# Autodesk Inventor assembly: Robot - Blue Alliance
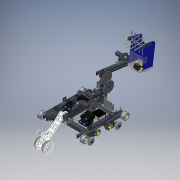
[picture p0: Inventor's stored thumbnail of the model, 180x180]
Saved by Autodesk Inventor 2016 (Build 200138000, 138)
## iProperties
Created: 2015-12-13
Part Number: Robot - Blue Alliance
Document SubType Name: Assembly
Designer: tbloo
Author: tbloo
## Documents named in this file (39)
- C:\Users\TimB\Documents\GitHub\phi_robotics\3d-models\FTC_Tetrix_KOP_Block_Party\Tim Bloot Designs\JAr JaR Bot\Robot - Blue Alliance.iam
- C:\Users\TimB\Documents\GitHub\phi_robotics\3d-models\FTC_Tetrix_KOP_Block_Party\Tim Bloot Designs\Base Plate.ipt
- C:\Users\TimB\Documents\GitHub\phi_robotics\3d-models\FTC_Tetrix_KOP_Block_Party\Tetrix_Kit_FTC\Autodesk Inventor Files\tetrix_c_channel-3.ipt
- C:\Users\TimB\Documents\GitHub\phi_robotics\3d-models\FTC_Tetrix_KOP_Block_Party\Tetrix_Kit_FTC\Autodesk Inventor Files\tetrix_c_channel-2.ipt
- C:\Users\TimB\Documents\GitHub\phi_robotics\3d-models\FTC_Tetrix_KOP_Block_Party\Tetrix_Kit_FTC\Autodesk Inventor Files\tetrix_motor_mount-old.ipt
- C:\Users\TimB\Documents\GitHub\phi_robotics\3d-models\FTC_Tetrix_KOP_Block_Party\Tetrix_Kit_FTC\Autodesk Inventor Files\tetrix_motor.iam
- C:\Users\TimB\Documents\GitHub\phi_robotics\3d-models\FTC_Tetrix_KOP_Block_Party\Tetrix_Kit_FTC\Autodesk Inventor Files\tetrix_bushing.ipt
- C:\Users\TimB\Documents\GitHub\phi_robotics\3d-models\FTC_Tetrix_KOP_Block_Party\Tim Bloot Designs\JAr JaR Bot\Tread Wheel Assembly.iam
- C:\Users\TimB\Documents\GitHub\phi_robotics\3d-models\FTC_Tetrix_KOP_Block_Party\Tetrix_Kit_FTC\Autodesk Inventor Files\tetrix_motor_controller.ipt
- C:\Users\TimB\Documents\GitHub\phi_robotics\3d-models\FTC_Tetrix_KOP_Block_Party\Tetrix_Kit_FTC\Autodesk Inventor Files\tetrix_c_channel-round.ipt
- C:\Users\TimB\Documents\GitHub\phi_robotics\3d-models\FTC_Tetrix_KOP_Block_Party\Tetrix_Kit_FTC\Autodesk Inventor Files\tetrix_c_channel-1.ipt
- C:\Users\TimB\Documents\GitHub\phi_robotics\3d-models\FTC_Tetrix_KOP_Block_Party\Tim Bloot Designs\JAr JaR Bot\Tread Sproket Gear Assembly 2.iam
- C:\Users\TimB\Documents\GitHub\phi_robotics\3d-models\FTC_Tetrix_KOP_Block_Party\Tim Bloot Designs\JAr JaR Bot\Motor Med Chain gear.iam
- C:\Users\TimB\Documents\GitHub\phi_robotics\3d-models\FTC_Tetrix_KOP_Block_Party\Tim Bloot Designs\JAr JaR Bot\tetrix_angle-144 MM.ipt
- C:\Users\TimB\Documents\GitHub\phi_robotics\3d-models\FTC_Tetrix_KOP_Block_Party\Tim Bloot Designs\JAr JaR Bot\inside Angle beam.ipt
- C:\Users\TimB\Documents\GitHub\phi_robotics\3d-models\FTC_Tetrix_KOP_Block_Party\Tetrix_Kit_FTC\Autodesk Inventor Files\tetrix_739107_2013.ipt
- C:\Users\TimB\Documents\GitHub\phi_robotics\3d-models\FTC_Tetrix_KOP_Block_Party\Tim Bloot Designs\JAr JaR Bot\cut c channel.ipt
- C:\Users\TimB\Documents\GitHub\phi_robotics\3d-models\FTC_Tetrix_KOP_Block_Party\Tetrix_Kit_FTC\Autodesk Inventor Files\tetrix_c_channel-4.ipt
- C:\Users\TimB\Documents\GitHub\phi_robotics\3d-models\FTC_Tetrix_KOP_Block_Party\Tetrix_Kit_FTC\Autodesk Inventor Files\tetrix_inside_corner_bracket.ipt
- C:\Users\TimB\Documents\GitHub\phi_robotics\3d-models\FTC_Tetrix_KOP_Block_Party\Tetrix_Kit_FTC\Autodesk Inventor Files\tetrix_worm_gear-p3.ipt
- C:\Users\TimB\Documents\GitHub\phi_robotics\3d-models\FTC_Tetrix_KOP_Block_Party\Tetrix_Kit_FTC\Autodesk Inventor Files\tetrix_servo_controller.ipt
- C:\Users\TimB\Documents\GitHub\phi_robotics\3d-models\FTC_Tetrix_KOP_Block_Party\Tim Bloot Designs\JAr JaR Bot\Blue Alliance Arm.iam
- C:\Users\TimB\Documents\GitHub\phi_robotics\3d-models\FTC_Tetrix_KOP_Block_Party\Tetrix_Kit_FTC\Autodesk Inventor Files\tetrix_standoff_post-1in.ipt
- C:\Users\TimB\Documents\GitHub\phi_robotics\3d-models\FTC_Tetrix_KOP_Block_Party\Tetrix_Kit_FTC\Autodesk Inventor Files\tetrix_axle_lock.iam
- C:\Users\TimB\Documents\GitHub\phi_robotics\3d-models\FTC_Tetrix_KOP_Block_Party\Tetrix_Kit_FTC\Autodesk Inventor Files\tetrix_gear-large.ipt
- C:\Users\TimB\Documents\GitHub\phi_robotics\3d-models\FTC_Tetrix_KOP_Block_Party\Tetrix_Kit_FTC\Autodesk Inventor Files\tetrix_gear-small.ipt
- C:\Users\TimB\Documents\GitHub\phi_robotics\3d-models\FTC_Tetrix_KOP_Block_Party\Tetrix_Kit_FTC\Autodesk Inventor Files\tetrix_axle_spacer_mount.ipt
- C:\Users\TimB\Documents\GitHub\phi_robotics\3d-models\FTC_Tetrix_KOP_Block_Party\Tetrix_Kit_FTC\Autodesk Inventor Files\tetrix_axle.ipt
- C:\Users\TimB\Documents\GitHub\phi_robotics\3d-models\FTC_Tetrix_KOP_Block_Party\Tetrix_Kit_FTC\Autodesk Inventor Files\tetrix_739092_2012.iam
- C:\Users\TimB\Documents\GitHub\phi_robotics\3d-models\FTC_Tetrix_KOP_Block_Party\Tetrix_Kit_FTC\Autodesk Inventor Files\tetrix_gear-med.ipt
- C:\Users\TimB\Documents\GitHub\phi_robotics\3d-models\FTC_Tetrix_KOP_Block_Party\Tim Bloot Designs\JAr JaR Bot\WheelieBar Blue Alliance.iam
- C:\Users\TimB\Documents\GitHub\phi_robotics\3d-models\FTC_Tetrix_KOP_Block_Party\Tetrix_Kit_FTC\Autodesk Inventor Files\tetrix_chain_gear-16t.ipt
- C:\Users\TimB\Documents\GitHub\phi_robotics\3d-models\FTC_Tetrix_KOP_Block_Party\Tetrix_Kit_FTC\Autodesk Inventor Files\tetrix_maxle_lock.iam
- C:\Users\TimB\Documents\GitHub\phi_robotics\3d-models\FTC_Tetrix_KOP_Block_Party\Tim Bloot Designs\Legacy Module.ipt
- C:\Users\TimB\Documents\GitHub\phi_robotics\3d-models\FTC_Tetrix_KOP_Block_Party\Tetrix_Kit_FTC\Autodesk Inventor Files\tetrix_batterypack.ipt
- C:\Users\TimB\Documents\GitHub\phi_robotics\3d-models\FTC_Tetrix_KOP_Block_Party\Tim Bloot Designs\Flag Mount.ipt
- C:\Users\TimB\Documents\GitHub\phi_robotics\3d-models\FTC_Tetrix_KOP_Block_Party\Tim Bloot Designs\Phone Mount 2.ipt
- C:\Users\TimB\Documents\GitHub\phi_robotics\3d-models\FTC_Tetrix_KOP_Block_Party\Tetrix_Kit_FTC\Autodesk Inventor Files\tetrix_739280_2013.ipt
- C:\Users\TimB\Documents\GitHub\phi_robotics\3d-models\FTC_Tetrix_KOP_Block_Party\Tetrix_Kit_FTC\Autodesk Inventor Files\tetrix_servo_body.ipt
## Components (128 placed, 38 different names)
1. Base Plate:1 — Rigid:117, Rigid:121, Rigid:127, Rigid:137, Rigid:140, Rigid:157, Rigid:162, Rigid:161, Rigid:163, Rigid:164, Mate:1
2. tetrix_c_channel-3:4 — Rigid:110, Rigid:122, Rigid:126, Rigid:142, Rigid:160
3. tetrix_c_channel-2:13 — Rigid:64, Rigid:111, Rigid:141
4. tetrix_c_channel-2:15 — Rigid:109, Rigid:143, Rigid:191
5. tetrix_c_channel-2:16 — Rigid:124, Rigid:148
6. tetrix_motor_mount-old:6
7. tetrix_motor:5 [sub-assembly] — Rigid:91
8. Tread Wheel Assembly:5 [sub-assembly]
9. Tread Wheel Assembly:6 [sub-assembly]
10. tetrix_c_channel-round:1 — Rigid:64, Rigid:65
11. tetrix_c_channel-1:1 — Rigid:65, Rotational:33, Rotational:34
12. tetrix_bushing:13 — Rotational:33, Rotational:42
13. tetrix_bushing:14 — Rotational:34
14. tetrix_c_channel-2:18 — Rigid:123, Rigid:125
15. tetrix_motor_mount-old:8 — Rotational:41
16. tetrix_c_channel-round:3
17. tetrix_c_channel-1:3
18. tetrix_bushing:17
19. tetrix_bushing:18 — Rotational:43
20. tetrix_motor:6 [sub-assembly] — Rotational:41, Rigid:92
21. Tread Sproket Gear Assembly 2:1 [sub-assembly] — Rotational:42
22. Tread Sproket Gear Assembly 2:2 [sub-assembly] — Rotational:43
23. Motor Med Chain gear:1 [sub-assembly] — Rigid:92
24. Motor Med Chain gear:2 [sub-assembly] — Rigid:91
25. tetrix_c_channel-3:5 — Rigid:116, Rigid:133, Rigid:136, Rigid:139
26. tetrix_c_channel-2:19 — Rigid:115, Rigid:135
27. tetrix_c_channel-2:20 — Rigid:134, Rigid:147
28. tetrix_c_channel-2:21 — Rigid:131, Rigid:144, Rigid:192
29. tetrix_motor_mount-old:9
30. tetrix_motor:7 [sub-assembly]
31. Tread Wheel Assembly:7 [sub-assembly]
32. Tread Wheel Assembly:8 [sub-assembly]
33. tetrix_c_channel-round:4
34. tetrix_c_channel-1:4
35. tetrix_bushing:19
36. tetrix_bushing:20
37. tetrix_c_channel-2:22 — Rigid:132, Rigid:138
38. tetrix_motor_mount-old:10
39. tetrix_c_channel-round:5
40. tetrix_c_channel-1:5
41. tetrix_bushing:21
42. tetrix_bushing:22
43. tetrix_motor:8 [sub-assembly]
44. Tread Sproket Gear Assembly 2:3 [sub-assembly]
45. Tread Sproket Gear Assembly 2:4 [sub-assembly]
46. Motor Med Chain gear:3 [sub-assembly]
47. Motor Med Chain gear:4 [sub-assembly]
48. tetrix_angle-144 MM:1 — Rigid:109, Rigid:110, Rigid:111
49. inside Angle beam:1 — Rigid:137, Rigid:138, Rigid:139
50. inside Angle beam:2 — Rigid:115, Rigid:116, Rigid:117
51. inside Angle beam:3 — Rigid:140, Rigid:141, Rigid:142, Mate:2
52. inside Angle beam:4 — Rigid:121, Rigid:122, Rigid:123
53. tetrix_angle-144 MM:2 — Rigid:124, Rigid:125, Rigid:126
54. tetrix_739107_2013:1 — Rigid:129
55. tetrix_739107_2013:2 — Rigid:128, Rigid:130
56. tetrix_motor_controller:1 — Rigid:127, Rigid:128, Rigid:129
57. tetrix_motor_controller:2 — Rigid:130
58. tetrix_angle-144 MM:3 — Rigid:134, Rigid:135, Rigid:136
59. tetrix_angle-144 MM:4 — Rigid:131, Rigid:132, Rigid:133
60. cut c channel:1 — Rigid:149, Rigid:151, Rigid:152, Rigid:172, Rotational:61, Rotational:62, Rotational:66, Rotational:67, Rigid:182, Rotational:75
61. cut c channel:2 — Rigid:143, Rigid:144, Rigid:151, Rigid:153, Mate:3, Rigid:188
62. tetrix_c_channel-4:1 — Rigid:145, Rigid:146, Rigid:150
63. tetrix_inside_corner_bracket:1 — Rigid:145, Rigid:148
64. tetrix_inside_corner_bracket:2 — Rigid:146, Rigid:147
65. tetrix_worm_gear-p3:1 — Rigid:149, Rigid:150
66. tetrix_c_channel-4:2 — Rigid:152, Rigid:153, Rotational:54, Rotational:55, Rotational:58, Rotational:59, Rigid:171, Rigid:189
67. tetrix_739107_2013:3 — Rigid:158
68. tetrix_739107_2013:4 — Rigid:159
69. tetrix_motor_controller:3 — Rigid:157
70. tetrix_servo_controller:1 — Rigid:158, Rigid:159
71. Blue Alliance Arm:1 [sub-assembly] — Rigid:186
72. tetrix_c_channel-1:6 — Rigid:160
73. tetrix_standoff_post-1in:1 — Rigid:162
74. tetrix_standoff_post-1in:2 — Rigid:163, Rigid:187
75. tetrix_standoff_post-1in:3 — Rigid:164
76. tetrix_standoff_post-1in:4 — Rigid:161
77. tetrix_bushing:23 — Rotational:54
78. tetrix_bushing:24 — Rotational:55, Rotational:56
79. tetrix_axle_lock:1 [sub-assembly] — Rigid:165, Rotational:56
80. tetrix_gear-large:1 — Rigid:165, Rigid:186
81. tetrix_gear-large:2 — Rigid:166
82. tetrix_gear-small:1 — Rigid:167, Rigid:168
83. tetrix_axle_spacer_mount:1 — Rigid:166, Rigid:167, Rotational:57
84. tetrix_axle_lock:2 [sub-assembly] — Rigid:168, Rigid:170
85. tetrix_bushing:25 — Rotational:57
86. tetrix_bushing:26 — Rotational:58
87. tetrix_bushing:27 — Rotational:59, Rotational:60
88. tetrix_axle:1 — Rigid:169, Rigid:170
89. tetrix_739092_2012:1 [sub-assembly] — Rigid:169, Rotational:60
90. tetrix_motor_mount-old:11 — Rigid:171, Rotational:64
91. tetrix_motor_mount-old:12 — Rigid:173, Rotational:65
92. tetrix_c_channel-round:6 — Rigid:172, Rigid:173
93. tetrix_gear-large:3 — Rigid:177
94. tetrix_axle_spacer_mount:2 — Rigid:175, Rigid:176
95. tetrix_gear-med:1 — Rigid:175
96. tetrix_bushing:28 — Rigid:176, Rigid:179
97. tetrix_739092_2012:2 [sub-assembly] — Rigid:178, Rigid:179
98. tetrix_axle_lock:3 [sub-assembly] — Rigid:177, Rotational:63
99. tetrix_axle:2 — Rigid:178, Rigid:180
100. tetrix_bushing:29 — Rotational:62
101. tetrix_bushing:30 — Rotational:61, Rotational:63
102. tetrix_739092_2012:3 [sub-assembly] — Rigid:180
103. tetrix_motor:9 [sub-assembly] — Rotational:64
104. tetrix_motor:10 [sub-assembly] — Rotational:65
105. tetrix_bushing:31 — Rotational:67, Rotational:70
106. tetrix_bushing:32 — Rotational:66
107. tetrix_c_channel-round:7 — Rigid:182, Rigid:183
108. tetrix_motor_mount-old:13 — Rigid:183, Rotational:69
109. tetrix_motor:11 [sub-assembly] — Rotational:69, Rigid:185
110. tetrix_maxle_lock:1 [sub-assembly] — Rigid:185, Rigid:194
111. WheelieBar Blue Alliance:1 [sub-assembly] — Rotational:70
112. Legacy Module:1 — Rigid:187
113. tetrix_batterypack:1 — Mate:1, Mate:2, Mate:3
114. Flag Mount:1 — Rigid:190
115. Phone Mount 2:1 — Rigid:188
116. tetrix_c_channel-1:7 — Rigid:189, Rigid:190
117. tetrix_739280_2013:1 — Rigid:191, Rotational:72, Rigid:193
118. tetrix_739280_2013:2 — Rigid:192, Rotational:71
119. tetrix_bushing:33 — Rotational:71
120. tetrix_bushing:34 — Rotational:72
121. tetrix_servo_body:1 — Rigid:193
122. tetrix_gear-small:2 — Rigid:194
123. tetrix_gear-med:3
124. tetrix_chain_gear-16t:2
125. tetrix_axle_lock:4 [sub-assembly]
126. tetrix_axle:3
127. tetrix_bushing:35
128. tetrix_bushing:36 — Rotational:75
## Relationships (140: WeldJoint 96, RevoluteJoint 41, Mate 3)
- [WeldJoint]: tetrix_c_channel-2:13 ↔ tetrix_motor_mount-old:6
- [RevoluteJoint]: tetrix_motor_mount-old:6 ↔ tetrix_motor:5
- [RevoluteJoint]: tetrix_c_channel-2:15 ↔ Tread Wheel Assembly:5
- [RevoluteJoint]: tetrix_c_channel-2:16 ↔ Tread Wheel Assembly:6
- Rigid:64 [WeldJoint]: tetrix_c_channel-2:13 ↔ tetrix_c_channel-round:1
- Rigid:65 [WeldJoint]: tetrix_c_channel-round:1 ↔ tetrix_c_channel-1:1
- Rotational:33 [RevoluteJoint]: tetrix_c_channel-1:1 ↔ tetrix_bushing:13
- Rotational:34 [RevoluteJoint]: tetrix_c_channel-1:1 ↔ tetrix_bushing:14
- [WeldJoint]: tetrix_c_channel-2:18 ↔ tetrix_motor_mount-old:8
- [WeldJoint]: tetrix_c_channel-2:18 ↔ tetrix_c_channel-round:3
- [WeldJoint]: tetrix_c_channel-round:3 ↔ tetrix_c_channel-1:3
- [RevoluteJoint]: tetrix_c_channel-1:3 ↔ tetrix_bushing:17
- [RevoluteJoint]: tetrix_c_channel-1:3 ↔ tetrix_bushing:18
- Rotational:41 [RevoluteJoint]: tetrix_motor_mount-old:8 ↔ tetrix_motor:6
- Rotational:42 [RevoluteJoint]: tetrix_bushing:13 ↔ Tread Sproket Gear Assembly 2:1
- Rotational:43 [RevoluteJoint]: tetrix_bushing:18 ↔ Tread Sproket Gear Assembly 2:2
- Rigid:91 [WeldJoint]: tetrix_motor:5 ↔ Motor Med Chain gear:2
- Rigid:92 [WeldJoint]: tetrix_motor:6 ↔ Motor Med Chain gear:1
- [WeldJoint]: tetrix_c_channel-2:19 ↔ tetrix_motor_mount-old:9
- [RevoluteJoint]: tetrix_motor_mount-old:9 ↔ tetrix_motor:7
- [RevoluteJoint]: tetrix_c_channel-2:20 ↔ Tread Wheel Assembly:7
- [RevoluteJoint]: tetrix_c_channel-2:21 ↔ Tread Wheel Assembly:8
- [WeldJoint]: tetrix_c_channel-2:19 ↔ tetrix_c_channel-round:4
- [WeldJoint]: tetrix_c_channel-round:4 ↔ tetrix_c_channel-1:4
- [RevoluteJoint]: tetrix_c_channel-1:4 ↔ tetrix_bushing:19
- [RevoluteJoint]: tetrix_c_channel-1:4 ↔ tetrix_bushing:20
- [WeldJoint]: tetrix_c_channel-2:22 ↔ tetrix_motor_mount-old:10
- [WeldJoint]: tetrix_c_channel-2:22 ↔ tetrix_c_channel-round:5
- [WeldJoint]: tetrix_c_channel-round:5 ↔ tetrix_c_channel-1:5
- [RevoluteJoint]: tetrix_c_channel-1:5 ↔ tetrix_bushing:21
- [RevoluteJoint]: tetrix_c_channel-1:5 ↔ tetrix_bushing:22
- [RevoluteJoint]: tetrix_motor_mount-old:10 ↔ tetrix_motor:8
- [RevoluteJoint]: tetrix_bushing:19 ↔ Tread Sproket Gear Assembly 2:3
- [RevoluteJoint]: tetrix_bushing:22 ↔ Tread Sproket Gear Assembly 2:4
- [WeldJoint]: tetrix_motor:7 ↔ Motor Med Chain gear:4
- [WeldJoint]: tetrix_motor:8 ↔ Motor Med Chain gear:3
- Rigid:109 [WeldJoint]: tetrix_c_channel-2:15 ↔ tetrix_angle-144 MM:1
- Rigid:110 [WeldJoint]: tetrix_c_channel-3:4 ↔ tetrix_angle-144 MM:1
- Rigid:111 [WeldJoint]: tetrix_c_channel-2:13 ↔ tetrix_angle-144 MM:1
- Rigid:115 [WeldJoint]: tetrix_c_channel-2:19 ↔ inside Angle beam:2
- Rigid:116 [WeldJoint]: tetrix_c_channel-3:5 ↔ inside Angle beam:2
- Rigid:117 [WeldJoint]: Base Plate:1 ↔ inside Angle beam:2
- Rigid:121 [WeldJoint]: Base Plate:1 ↔ inside Angle beam:4
- Rigid:122 [WeldJoint]: tetrix_c_channel-3:4 ↔ inside Angle beam:4
- Rigid:123 [WeldJoint]: tetrix_c_channel-2:18 ↔ inside Angle beam:4
- Rigid:124 [WeldJoint]: tetrix_c_channel-2:16 ↔ tetrix_angle-144 MM:2
- Rigid:125 [WeldJoint]: tetrix_c_channel-2:18 ↔ tetrix_angle-144 MM:2
- Rigid:126 [WeldJoint]: tetrix_c_channel-3:4 ↔ tetrix_angle-144 MM:2
- Rigid:127 [WeldJoint]: Base Plate:1 ↔ tetrix_motor_controller:1
- Rigid:128 [WeldJoint]: tetrix_739107_2013:2 ↔ tetrix_motor_controller:1
- Rigid:129 [WeldJoint]: tetrix_739107_2013:1 ↔ tetrix_motor_controller:1
- Rigid:130 [WeldJoint]: tetrix_739107_2013:2 ↔ tetrix_motor_controller:2
- Rigid:131 [WeldJoint]: tetrix_c_channel-2:21 ↔ tetrix_angle-144 MM:4
- Rigid:132 [WeldJoint]: tetrix_c_channel-2:22 ↔ tetrix_angle-144 MM:4
- Rigid:133 [WeldJoint]: tetrix_c_channel-3:5 ↔ tetrix_angle-144 MM:4
- Rigid:134 [WeldJoint]: tetrix_c_channel-2:20 ↔ tetrix_angle-144 MM:3
- Rigid:135 [WeldJoint]: tetrix_c_channel-2:19 ↔ tetrix_angle-144 MM:3
- Rigid:136 [WeldJoint]: tetrix_c_channel-3:5 ↔ tetrix_angle-144 MM:3
- Rigid:137 [WeldJoint]: Base Plate:1 ↔ inside Angle beam:1
- Rigid:138 [WeldJoint]: tetrix_c_channel-2:22 ↔ inside Angle beam:1
- Rigid:139 [WeldJoint]: tetrix_c_channel-3:5 ↔ inside Angle beam:1
- Rigid:140 [WeldJoint]: Base Plate:1 ↔ inside Angle beam:3
- Rigid:141 [WeldJoint]: tetrix_c_channel-2:13 ↔ inside Angle beam:3
- Rigid:142 [WeldJoint]: tetrix_c_channel-3:4 ↔ inside Angle beam:3
- Rigid:143 [WeldJoint]: tetrix_c_channel-2:15 ↔ cut c channel:2
- Rigid:144 [WeldJoint]: tetrix_c_channel-2:21 ↔ cut c channel:2
- Rigid:145 [WeldJoint]: tetrix_c_channel-4:1 ↔ tetrix_inside_corner_bracket:1
- Rigid:146 [WeldJoint]: tetrix_c_channel-4:1 ↔ tetrix_inside_corner_bracket:2
- Rigid:147 [WeldJoint]: tetrix_c_channel-2:20 ↔ tetrix_inside_corner_bracket:2
- Rigid:148 [WeldJoint]: tetrix_c_channel-2:16 ↔ tetrix_inside_corner_bracket:1
- Rigid:149 [WeldJoint]: cut c channel:1 ↔ tetrix_worm_gear-p3:1
- Rigid:150 [WeldJoint]: tetrix_c_channel-4:1 ↔ tetrix_worm_gear-p3:1
- Rigid:151 [WeldJoint]: cut c channel:1 ↔ cut c channel:2
- Rigid:152 [WeldJoint]: cut c channel:1 ↔ tetrix_c_channel-4:2
- Rigid:153 [WeldJoint]: cut c channel:2 ↔ tetrix_c_channel-4:2
- [WeldJoint]: tetrix_739107_2013:4 ↔ tetrix_motor_controller:3
- [WeldJoint]: tetrix_739107_2013:3 ↔ tetrix_motor_controller:3
- Rigid:157 [WeldJoint]: Base Plate:1 ↔ tetrix_motor_controller:3
- Rigid:158 [WeldJoint]: tetrix_739107_2013:3 ↔ tetrix_servo_controller:1
- Rigid:159 [WeldJoint]: tetrix_739107_2013:4 ↔ tetrix_servo_controller:1
- Rigid:160 [WeldJoint]: tetrix_c_channel-3:4 ↔ tetrix_c_channel-1:6
- Rigid:162 [WeldJoint]: Base Plate:1 ↔ tetrix_standoff_post-1in:1
- Rigid:161 [WeldJoint]: Base Plate:1 ↔ tetrix_standoff_post-1in:4
- Rigid:163 [WeldJoint]: Base Plate:1 ↔ tetrix_standoff_post-1in:2
- Rigid:164 [WeldJoint]: Base Plate:1 ↔ tetrix_standoff_post-1in:3
- Rotational:54 [RevoluteJoint]: tetrix_c_channel-4:2 ↔ tetrix_bushing:23
- Rotational:55 [RevoluteJoint]: tetrix_c_channel-4:2 ↔ tetrix_bushing:24
- Rigid:165 [WeldJoint]: tetrix_axle_lock:1 ↔ tetrix_gear-large:1
- Rotational:56 [RevoluteJoint]: tetrix_bushing:24 ↔ tetrix_axle_lock:1
- Rigid:166 [WeldJoint]: tetrix_gear-large:2 ↔ tetrix_axle_spacer_mount:1
- Rigid:167 [WeldJoint]: tetrix_gear-small:1 ↔ tetrix_axle_spacer_mount:1
- Rotational:57 [RevoluteJoint]: tetrix_axle_spacer_mount:1 ↔ tetrix_bushing:25
- Rigid:168 [WeldJoint]: tetrix_gear-small:1 ↔ tetrix_axle_lock:2
- Rotational:58 [RevoluteJoint]: tetrix_c_channel-4:2 ↔ tetrix_bushing:26
- Rotational:59 [RevoluteJoint]: tetrix_c_channel-4:2 ↔ tetrix_bushing:27
- Rigid:169 [WeldJoint]: tetrix_axle:1 ↔ tetrix_739092_2012:1
- Rotational:60 [RevoluteJoint]: tetrix_bushing:27 ↔ tetrix_739092_2012:1
- Rigid:170 [WeldJoint] (-41.4 mm): tetrix_axle_lock:2 ↔ tetrix_axle:1
- Rigid:171 [WeldJoint]: tetrix_c_channel-4:2 ↔ tetrix_motor_mount-old:11
- Rigid:172 [WeldJoint]: cut c channel:1 ↔ tetrix_c_channel-round:6
- Rigid:173 [WeldJoint]: tetrix_motor_mount-old:12 ↔ tetrix_c_channel-round:6
- [WeldJoint]: tetrix_gear-large:3 ↔ tetrix_axle_spacer_mount:2
- Rigid:175 [WeldJoint]: tetrix_axle_spacer_mount:2 ↔ tetrix_gear-med:1
- Rigid:176 [WeldJoint]: tetrix_axle_spacer_mount:2 ↔ tetrix_bushing:28
- Rigid:177 [WeldJoint]: tetrix_gear-large:3 ↔ tetrix_axle_lock:3
- Rigid:178 [WeldJoint]: tetrix_739092_2012:2 ↔ tetrix_axle:2
- Rigid:179 [WeldJoint]: tetrix_bushing:28 ↔ tetrix_739092_2012:2
- Rotational:61 [RevoluteJoint]: cut c channel:1 ↔ tetrix_bushing:30
- Rotational:62 [RevoluteJoint]: cut c channel:1 ↔ tetrix_bushing:29
- Rotational:63 [RevoluteJoint]: tetrix_axle_lock:3 ↔ tetrix_bushing:30
- Rigid:180 [WeldJoint] (-17.713 mm): tetrix_axle:2 ↔ tetrix_739092_2012:3
- Rotational:64 [RevoluteJoint]: tetrix_motor_mount-old:11 ↔ tetrix_motor:9
- Rotational:65 [RevoluteJoint]: tetrix_motor_mount-old:12 ↔ tetrix_motor:10
- Rotational:66 [RevoluteJoint]: cut c channel:1 ↔ tetrix_bushing:32
- Rotational:67 [RevoluteJoint]: cut c channel:1 ↔ tetrix_bushing:31
- Rigid:182 [WeldJoint]: cut c channel:1 ↔ tetrix_c_channel-round:7
- Rigid:183 [WeldJoint]: tetrix_c_channel-round:7 ↔ tetrix_motor_mount-old:13
- Rotational:69 [RevoluteJoint]: tetrix_motor_mount-old:13 ↔ tetrix_motor:11
- Rigid:185 [WeldJoint] (-5 mm): tetrix_motor:11 ↔ tetrix_maxle_lock:1
- Rigid:186 [WeldJoint] (6.35 mm): Blue Alliance Arm:1 ↔ tetrix_gear-large:1
- Rotational:70 [RevoluteJoint]: tetrix_bushing:31 ↔ WheelieBar Blue Alliance:1
- Rigid:187 [WeldJoint]: tetrix_standoff_post-1in:2 ↔ Legacy Module:1
- Mate:1: Base Plate:1 ↔ tetrix_batterypack:1
- Mate:2 (3 mm): inside Angle beam:3 ↔ tetrix_batterypack:1
- Mate:3 (3 mm): cut c channel:2 ↔ tetrix_batterypack:1
- Rigid:188 [WeldJoint]: cut c channel:2 ↔ Phone Mount 2:1
- Rigid:189 [WeldJoint]: tetrix_c_channel-4:2 ↔ tetrix_c_channel-1:7
- Rigid:190 [WeldJoint]: Flag Mount:1 ↔ tetrix_c_channel-1:7
- Rigid:191 [WeldJoint]: tetrix_c_channel-2:15 ↔ tetrix_739280_2013:1
- Rigid:192 [WeldJoint]: tetrix_c_channel-2:21 ↔ tetrix_739280_2013:2
- Rotational:71 [RevoluteJoint]: tetrix_739280_2013:2 ↔ tetrix_bushing:33
- Rotational:72 [RevoluteJoint]: tetrix_739280_2013:1 ↔ tetrix_bushing:34
- Rigid:193 [WeldJoint]: tetrix_739280_2013:1 ↔ tetrix_servo_body:1
- Rigid:194 [WeldJoint]: tetrix_maxle_lock:1 ↔ tetrix_gear-small:2
- [WeldJoint]: tetrix_gear-med:3 ↔ tetrix_axle_lock:4
- [WeldJoint]: tetrix_gear-med:3 ↔ tetrix_chain_gear-16t:2
- [WeldJoint]: tetrix_axle_lock:4 ↔ tetrix_axle:3
- [RevoluteJoint]: tetrix_chain_gear-16t:2 ↔ tetrix_bushing:35
- [RevoluteJoint]: tetrix_bushing:35 ↔ tetrix_bushing:36
- Rotational:75 [RevoluteJoint]: cut c channel:1 ↔ tetrix_bushing:36
## Named parameters: d112_d58_d39 = 0 mm, d113_d59_d40 = -5.431137 deg, d114_d60_d41 = 0 mm, d115_d61_d42 = 0.840635 deg, d116_d65_d11 = 0 mm, d122_d71_d21 = 0 mm, d123_d72_d22 = -45.624239 deg, d153_d150_d116_d65_d11 = 0 mm, d154_d143_d137 = 0 mm, d155_d144_d138 = 0 mm, d156_d145_d139 = 0 mm, d157_d146_d140 = 0 deg, d158_d147_d141 = 0 mm, d159_d148_d142 = 0 deg, d210_d112_d58_d39 = 0 mm, d211_d113_d59_d40 = -5.431137 deg, d212_d170 = 0 mm, d213_d171 = 0 deg, d219_d208 = 0 mm, d220_d209 = 0 mm, d221_d137 = 0 mm, d222_d138 = 0 mm, d223_d139 = 0 mm, d224_d140 = 0.202797 deg, d225_d141 = 0 mm, d226_d142 = 0 deg, d227_d153_d150_d116_d65_d11 = 0 mm, d228_d154_d143_d137 = 0 mm, d229_d155_d144_d138 = 0 mm, d230_d156_d145_d139 = 0 mm, d231_d157_d146_d140 = 0 deg, d232_d158_d147_d141 = 0 mm, d233_d159_d148_d142 = 0 deg, d236_d166 = 0 mm, d237_d167 = -134.685077 deg, d238_d168 = 0 mm, d239_d169 = -0.202797 deg, d240_d114_d60_d41 = 0 mm, d241_d115_d61_d42 = 0.840635 deg, d242_d116_d65_d11 = 0 mm, d243_d122_d71_d21 = 0 mm, d244_d123_d72_d22 = -50.322066 deg, d295_d269 = 0 mm, d296_d270 = 0 mm, d330_d314 = 0 mm, d387_d370 = 0 mm, d388_d371 = 0 mm
